# Autodesk Inventor assembly: Botonera_petit
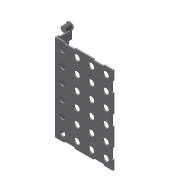
[picture p0: Inventor's stored thumbnail of the model, 180x180]
Saved by Autodesk Inventor 2017 (Build 210142000, 142)
## iProperties
Created: 2017-06-21
Part Number: Botonera_petit
Document SubType Name: Assembly
Designer: Butri
Author: Butri
## Documents named in this file (4)
- D:\Google Drive\Proyectil\Proyectos\Internos _ 2017\Botones\MatrizBotones_3\Botonera_petit.iam
- D:\Google Drive\Proyectil\Proyectos\Internos _ 2017\Botones\MatrizBotones_3\Base_modulos.ipt
- D:\Google Drive\Proyectil\Proyectos\Internos _ 2017\Botones\MatrizBotones_3\Boton.ipt
- D:\Google Drive\Proyectil\Proyectos\Internos _ 2017\Botones\MatrizBotones_3\Frontal.ipt
## Components (3 placed, 3 different names)
1. Base_modulos:1 — Flush:1
2. Boton:1
3. Frontal:1 — Flush:1
## Relationships (1: Flush 1)
- Flush:1: Base_modulos:1 ↔ Frontal:1
